# Autodesk Inventor assembly: insertAssembly-3
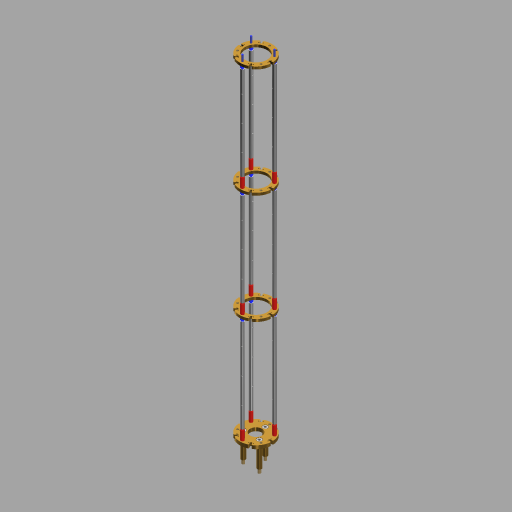
[picture p0: Inventor's stored thumbnail of the model, 512x512]
Saved by Autodesk Inventor 2024 (Build 280153020, 153B)
## iProperties
Created: 2023-09-24
Part Number: insertAssembly-3
Document SubType Name: Assembly
Designer: schanen
Author: schanen
## Documents named in this file (7)
- C:\Users\schanen\Documents\Inventor\he4inserts\insertAssembly-3.iam
- C:\Users\schanen\Documents\Inventor\he4inserts\Insert_flange.ipt
- C:\Users\schanen\Documents\Inventor\he4inserts\Insert_flange_Top.ipt
- C:\Users\schanen\Documents\Inventor\he4inserts\Screw_StainlessSteal_M3_SocketCap_6mm.ipt
- C:\Users\schanen\Documents\Inventor\he4inserts\Fitting-3.ipt
- C:\Users\schanen\Documents\Inventor\he4inserts\CompositeSupport-3.iam
- C:\Users\schanen\Documents\Inventor\he4inserts\Screw_StainlessSteal_M2_SocketCap_10mm.ipt
## Components (22 placed, 6 different names)
1. Insert_flange_Top:1 — Mate:1, Mate:2, Mate:3, Mate:4, Mate:6, Mate:7, Mate:9, Mate:11, Mate:12, Mate:13, Mate:14
2. Fitting-3:1 [sub-assembly] — Mate:2, Mate:11
3. Fitting-3:2
4. Fitting-3:3
5. Screw_StainlessSteal_M2_SocketCap_10mm:1 — Mate:13, Mate:14
6. Screw_StainlessSteal_M2_SocketCap_10mm:2
7. Screw_StainlessSteal_M2_SocketCap_10mm:3
8. Screw_StainlessSteal_M3_SocketCap_6mm:1 — Mate:1, Mate:12
9. Screw_StainlessSteal_M3_SocketCap_6mm:2
10. Screw_StainlessSteal_M3_SocketCap_6mm:3
11. Insert_flange:1 — Mate:6, Mate:8, Mate:10
12. Insert_flange:2
13. Insert_flange:3
14. CompositeSupport-3:1 [sub-assembly] — Mate:7, Mate:8, Mate:9, Mate:10
15. CompositeSupport-3:2 [sub-assembly]
16. CompositeSupport-3:3 [sub-assembly]
17. CompositeSupport-3:4 [sub-assembly]
18. CompositeSupport-3:5 [sub-assembly]
19. CompositeSupport-3:6 [sub-assembly]
20. CompositeSupport-3:7 [sub-assembly]
21. CompositeSupport-3:8 [sub-assembly]
22. CompositeSupport-3:9 [sub-assembly]
## Component patterns: (3 elements, first: Fitting-3:1), (3 elements, first: Screw_StainlessSteal_M2_SocketCap_10mm:1), (3 elements, first: Screw_StainlessSteal_M3_SocketCap_6mm:1), (3 elements, first: Insert_flange:1), (3 elements, first: CompositeSupport-3:1), Component Pattern 13:2 (3 elements), Component Pattern 13:3 (3 elements)
## Relationships (13: Mate 13)
- Mate:1: Insert_flange_Top:1 ↔ Screw_StainlessSteal_M3_SocketCap_6mm:1
- Mate:2: Insert_flange_Top:1 ↔ Fitting-3:1
- Mate:3: Insert_flange_Top:1
- Mate:4: Insert_flange_Top:1
- Mate:6: Insert_flange_Top:1 ↔ Insert_flange:1
- Mate:7: Insert_flange_Top:1 ↔ CompositeSupport-3:1
- Mate:8: Insert_flange:1 ↔ CompositeSupport-3:1
- Mate:9: Insert_flange_Top:1 ↔ CompositeSupport-3:1
- Mate:10: Insert_flange:1 ↔ CompositeSupport-3:1
- Mate:11: Insert_flange_Top:1 ↔ Fitting-3:1
- Mate:12: Insert_flange_Top:1 ↔ Screw_StainlessSteal_M3_SocketCap_6mm:1
- Mate:13: Insert_flange_Top:1 ↔ Screw_StainlessSteal_M2_SocketCap_10mm:1
- Mate:14: Insert_flange_Top:1 ↔ Screw_StainlessSteal_M2_SocketCap_10mm:1
